# Autodesk Inventor assembly: body
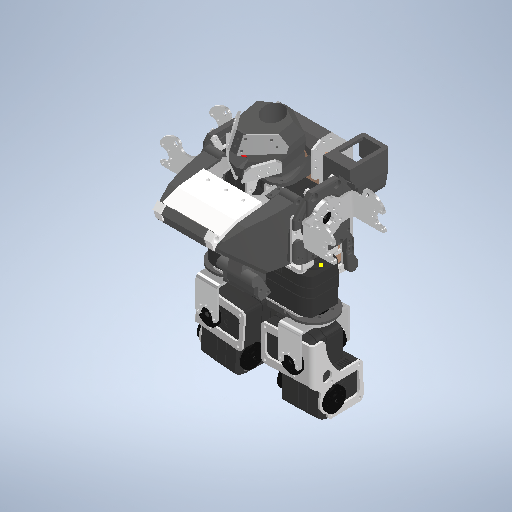
[picture p0: Inventor's stored thumbnail of the model, 512x512]
Saved by Autodesk Inventor 2026.1 (Build 301233020, 233B)
## iProperties
Created: 2024-10-10
Part Number: body
Document SubType Name: Assembly
Designer: hibik
Author: hibik
## Documents named in this file (6)
- C:\Users\hibik\Documents\Robomech\HR\Eglantyne_mark2\hard\body.iam
- C:\Users\hibik\Documents\Robomech\HR\Eglantyne_mark2\hard\under_body\under_body.iam
- C:\Users\hibik\Documents\Robomech\HR\Eglantyne_mark2\hard\needed_model\battely.ipt
- C:\Users\hibik\Documents\Robomech\HR\Eglantyne_mark2\hard\head\head.iam
- C:\Users\hibik\Documents\Robomech\HR\Eglantyne_mark2\hard\board\board.iam
- C:\Users\hibik\Documents\Robomech\HR\Eglantyne_mark2\hard\upper_body\upperbody.iam
## Components (5 placed, 5 different names)
1. under_body:1 [sub-assembly] — 挿入:1, 挿入:2
2. battely:1
3. board:1 [sub-assembly] — 挿入:1, 角度:3
4. upperbody:1 [sub-assembly] — 挿入:2, 角度:3
5. head:4 [sub-assembly]
## Relationships (3: Insert 2, Angle 1)
- 挿入:1 [Insert] (0.5 mm): under_body:1 ↔ board:1
- 挿入:2 [Insert]: under_body:1 ↔ upperbody:1
- 角度:3 [Angle] (0 deg): board:1 ↔ upperbody:1
